# Autodesk Inventor assembly: Ensamble MDF
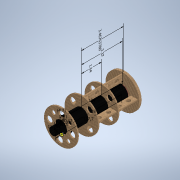
[picture p0: Inventor's stored thumbnail of the model, 180x180]
Saved by Autodesk Inventor 2020 (Build 240168000, 168)
## iProperties
Created: 2021-09-30
Part Number: Ensamble MDF
Document SubType Name: Assembly
Designer: Carlos
Mass: 117.714 g
Surface Area: 1062.22 cm^2
Volume: 127.325 cm^3
Density: 0.924516 g/cm^3
Author: Carlos
## Documents named in this file (6)
- \\CARLOS-PC\Shared\UdeA\Diseño Conceptual\CAD Cohete\CAD 2 - copia\Anillos\CAD\Ensamble MDF.iam
- \\CARLOS-PC\Shared\UdeA\Diseño Conceptual\CAD Cohete\Aerotech G80 7T\Aeoech G80 7T\G80.iam
- \\CARLOS-PC\Shared\UdeA\Diseño Conceptual\CAD Cohete\CAD 2 - copia\Anillos\CAD\MDF\Anillo de Centrado.ipt
- \\CARLOS-PC\Shared\UdeA\Diseño Conceptual\CAD Cohete\CAD 2 - copia\Anillos\CAD\MDF\Anillo de Empuje.ipt
- \\CARLOS-PC\Shared\UdeA\Diseño Conceptual\CAD Cohete\CAD 2 - copia\Anillos\CAD\MDF\Estructura Anillos.ipt
- \\CARLOS-PC\Shared\UdeA\Diseño Conceptual\CAD Cohete\CAD 2 - copia\Anillos\CAD\MDF\Anillo de Soporte.ipt
## Components (10 placed, 5 different names)
1. G80:1 [sub-assembly] — Mate:1, Mate:2, Mate:3, Mate:5, Mate:7, Mate:11, Mate:12
2. Anillo de Centrado:1 — Mate:1, Mate:6, Flush:1, Mate:15
3. Anillo de Empuje:1 — Mate:3, Mate:7, Mate:16, Mate:17
4. Anillo de Centrado:2 — Mate:2, Mate:5, Mate:6, Mate:13, Mate:14
5. Anillo de Soporte:1 — Mate:11, Mate:12
6. Anillo de Empuje:2 — Mate:16, Mate:17
7. Estructura Anillos:1 — Flush:1, Mate:13, Mate:14, Mate:15
8. Estructura Anillos:2
9. Estructura Anillos:3
10. Estructura Anillos:4
## Component patterns: (4 elements, first: Estructura Anillos:1)
## Relationships (14: Mate 13, Flush 1)
- Mate:1: G80:1 ↔ Anillo de Centrado:1
- Mate:2: G80:1 ↔ Anillo de Centrado:2
- Mate:3: G80:1 ↔ Anillo de Empuje:1
- Mate:5 (39.266 mm): G80:1 ↔ Anillo de Centrado:2
- Mate:6 (39.266 mm): Anillo de Centrado:1 ↔ Anillo de Centrado:2
- Mate:7: G80:1 ↔ Anillo de Empuje:1
- Flush:1: Anillo de Centrado:1 ↔ Estructura Anillos:1
- Mate:11: G80:1 ↔ Anillo de Soporte:1
- Mate:12: G80:1 ↔ Anillo de Soporte:1
- Mate:13: Anillo de Centrado:2 ↔ Estructura Anillos:1
- Mate:14: Anillo de Centrado:2 ↔ Estructura Anillos:1
- Mate:15: Anillo de Centrado:1 ↔ Estructura Anillos:1
- Mate:16: Anillo de Empuje:1 ↔ Anillo de Empuje:2
- Mate:17: Anillo de Empuje:1 ↔ Anillo de Empuje:2
